# Autodesk Inventor assembly: entero
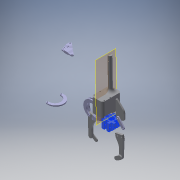
[picture p0: Inventor's stored thumbnail of the model, 180x180]
Saved by Autodesk Inventor 2018 (Build 220112000, 112)
## iProperties
Created: 2018-05-25
Part Number: entero
Document SubType Name: Assembly
Designer: vigus
Author: vigus
## Documents named in this file (7)
- C:\Users\vigus\Documents\gihug\hecatonquiros\cad_models\accesories\gripper\entero.iam
- C:\Users\vigus\Documents\gihug\hecatonquiros\cad_models\tools\gripper\serial_model_0dof\core_attachment.ipt
- C:\Users\vigus\Documents\gihug\hecatonquiros\cad_models\accesories\gripper\Imported Components\garra_pilar\garra_pilar.ipt
- C:\Users\vigus\Documents\gihug\hecatonquiros\cad_models\tools\gripper\serial_model_0dof\ScrewActuatorGripperCenter.ipt
- C:\Users\vigus\Documents\gihug\hecatonquiros\cad_models\tools\gripper\serial_model_0dof\gripper.ipt
- C:\Users\vigus\Documents\gihug\hecatonquiros\cad_models\accesories\gripper\garra_pilar_3.ipt
- C:\Users\vigus\Documents\gihug\hecatonquiros\cad_models\accesories\gripper\barra_tri.ipt
## Components (12 placed, 6 different names)
1. core_attachment:1 — Mate:2, Mate:3, Mate:13, Mate:14, Angle:1, Mate:32, Mate:42, Mate:43, Mate:52, Mate:53, Mate:55, Mate:56
2. garra_pilar:1 — Mate:2, Mate:3
3. ScrewActuatorGripperCenter:1 — Angle:1, Mate:32, Mate:58, Mate:59
4. garra_pilar:2 — Mate:13, Mate:14, Mate:62
5. gripper:1 — Mate:54, Mate:57, Mate:61
6. gripper:2
7. garra_pilar:3 — Mate:42, Mate:43, Mate:60
8. garra_pilar_3:2 — Mate:55, Mate:56, Mate:57
9. garra_pilar_3:3 — Mate:52, Mate:53, Mate:54
10. garra_pilar_3:4
11. barra_tri:1 — Mate:58, Mate:59, Mate:60, Mate:61, Mate:62
12. barra_tri:2
## Relationships (19: Mate 18, Angle 1)
- Mate:2: core_attachment:1 ↔ garra_pilar:1
- Mate:3: core_attachment:1 ↔ garra_pilar:1
- Mate:13: core_attachment:1 ↔ garra_pilar:2
- Mate:14: core_attachment:1 ↔ garra_pilar:2
- Angle:1 (0 deg): core_attachment:1 ↔ ScrewActuatorGripperCenter:1
- Mate:32: core_attachment:1 ↔ ScrewActuatorGripperCenter:1
- Mate:42: core_attachment:1 ↔ garra_pilar:3
- Mate:43: core_attachment:1 ↔ garra_pilar:3
- Mate:52: core_attachment:1 ↔ garra_pilar_3:3
- Mate:53: core_attachment:1 ↔ garra_pilar_3:3
- Mate:54: gripper:1 ↔ garra_pilar_3:3
- Mate:55: core_attachment:1 ↔ garra_pilar_3:2
- Mate:56: core_attachment:1 ↔ garra_pilar_3:2
- Mate:57: gripper:1 ↔ garra_pilar_3:2
- Mate:58: ScrewActuatorGripperCenter:1 ↔ barra_tri:1
- Mate:59: ScrewActuatorGripperCenter:1 ↔ barra_tri:1
- Mate:60: garra_pilar:3 ↔ barra_tri:1
- Mate:61: gripper:1 ↔ barra_tri:1
- Mate:62: garra_pilar:2 ↔ barra_tri:1
